# Autodesk Inventor assembly: Test Assembly
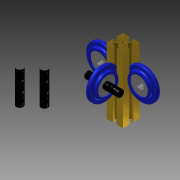
[picture p0: Inventor's stored thumbnail of the model, 180x180]
Saved by Autodesk Inventor 2014 (Build 180170000, 170)
## iProperties
Created: 2015-02-07
Part Number: Test Assembly
Document SubType Name: Assembly
Designer: Spooner
Author: Spooner
## Documents named in this file (6)
- C:\Users\Spooner\Documents\Inventor\80-20  Linear Bearing\Test Assembly.iam
- C:\Users\Spooner\Documents\Inventor\80-20  Linear Bearing\1_5 80-20 x 6in.ipt
- C:\Users\Spooner\Documents\Inventor\80-20  Linear Bearing\Big Bearing.ipt
- C:\Users\Spooner\Documents\Inventor\80-20  Linear Bearing\Big Bearing Cover.ipt
- C:\Users\Spooner\Documents\Inventor\80-20  Linear Bearing\Igus Rod.ipt
- C:\Users\Spooner\Documents\Inventor\80-20  Linear Bearing\Bearing-Axle Sleeve.ipt
## Components (14 placed, 5 different names)
1. 1_5 80-20 x 6in:1 — Mate:1, Mate:2, Mate:3, Mate:6, Flush:1, Flush:2
2. Big Bearing:1 — Mate:3, Mate:4, Mate:5, Flush:1, Flush:3, Mate:7
3. Big Bearing:2 — Mate:1, Mate:4, Flush:2, Insert:1
4. Big Bearing:3 — Mate:2, Mate:5, Mate:6, Insert:2
5. Big Bearing Cover:1 — Flush:3, Insert:4
6. Big Bearing Cover:2 — Insert:1, Insert:3
7. Big Bearing Cover:3 — Insert:2, Insert:5
8. Big Bearing Cover:4 — Insert:5
9. Big Bearing Cover:5 — Insert:4
10. Big Bearing Cover:6 — Insert:3
11. Igus Rod:1
12. Igus Rod:2
13. Igus Rod:3 — Mate:7, Flush:4
14. Bearing-Axle Sleeve:1 — Flush:4
## Relationships (16: Mate 7, Insert 5, Flush 4)
- Mate:1: 1_5 80-20 x 6in:1 ↔ Big Bearing:2
- Mate:2: 1_5 80-20 x 6in:1 ↔ Big Bearing:3
- Mate:3: 1_5 80-20 x 6in:1 ↔ Big Bearing:1
- Mate:4: Big Bearing:1 ↔ Big Bearing:2
- Mate:5: Big Bearing:1 ↔ Big Bearing:3
- Mate:6 (27.305 mm): 1_5 80-20 x 6in:1 ↔ Big Bearing:3
- Flush:1 (27.305 mm): 1_5 80-20 x 6in:1 ↔ Big Bearing:1
- Flush:2 (-27.305 mm): 1_5 80-20 x 6in:1 ↔ Big Bearing:2
- Flush:3: Big Bearing:1 ↔ Big Bearing Cover:1
- Insert:1: Big Bearing:2 ↔ Big Bearing Cover:2
- Insert:2: Big Bearing:3 ↔ Big Bearing Cover:3
- Insert:3: Big Bearing Cover:2 ↔ Big Bearing Cover:6
- Insert:4: Big Bearing Cover:1 ↔ Big Bearing Cover:5
- Insert:5: Big Bearing Cover:3 ↔ Big Bearing Cover:4
- Mate:7: Big Bearing:1 ↔ Igus Rod:3
- Flush:4: Igus Rod:3 ↔ Bearing-Axle Sleeve:1
